# Autodesk Inventor assembly: CN3065 Solar Charger board
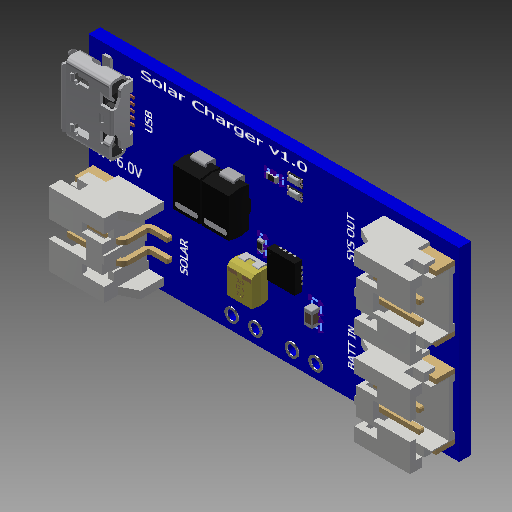
[picture p0: Inventor's stored thumbnail of the model, 512x512]
Saved by Autodesk Inventor 2018 (Build 220112000, 112)
## iProperties
Created: 2019-03-28
Part Number: CN3065 Solar Charger board
Document SubType Name: Assembly
Designer: ZEUSLAP
Author: ZEUSLAP
## Documents named in this file (11)
- C:\Users\ZEUSLAP\YandexDisk\Inventor\solar_harvester_145x145\parts\CN3065 Solar Charger board\CN3065 Solar Charger board.iam
- C:\Users\ZEUSLAP\YandexDisk\Inventor\solar_harvester_145x145\parts\CN3065 Solar Charger board\parts\board.ipt
- C:\Users\ZEUSLAP\YandexDisk\Inventor\solar_harvester_145x145\parts\CN3065 Solar Charger board\parts\micro USB.ipt
- C:\Users\ZEUSLAP\YandexDisk\Inventor\solar_harvester_145x145\parts\CN3065 Solar Charger board\parts\S2B-PH-SM4-TB.ipt
- C:\Users\ZEUSLAP\YandexDisk\Inventor\solar_harvester_145x145\parts\CN3065 Solar Charger board\parts\Diode SMA.ipt
- C:\Users\ZEUSLAP\YandexDisk\Inventor\solar_harvester_145x145\parts\CN3065 Solar Charger board\parts\Tant Cap SMD size B _ 3528-21.ipt
- C:\Users\ZEUSLAP\YandexDisk\Inventor\solar_harvester_145x145\parts\CN3065 Solar Charger board\parts\QFN-16 (3x3).ipt
- C:\Users\ZEUSLAP\YandexDisk\Inventor\solar_harvester_145x145\parts\CN3065 Solar Charger board\parts\CAPC-0603-T0.9-BN.ipt
- C:\Users\ZEUSLAP\YandexDisk\Inventor\solar_harvester_145x145\parts\CN3065 Solar Charger board\parts\RESC-0402.ipt
- C:\Users\ZEUSLAP\YandexDisk\Inventor\solar_harvester_145x145\parts\CN3065 Solar Charger board\parts\0603 LED v7.ipt
- C:\Users\ZEUSLAP\YandexDisk\Inventor\solar_harvester_145x145\parts\CN3065 Solar Charger board\parts\hole_plating.ipt
## Components (22 placed, 10 different names)
1. board:1 — Mate:4, Angle:1, Mate:7, Mate:8, Mate:9, Mate:10, Mate:11, Angle:2, Angle:3, Angle:4, Flush:1, Flush:2, Flush:3, Flush:4, Flush:5, Flush:6, Mate:12, Mate:13, Angle:5, Angle:6, Mate:14, Mate:15, Flush:7, Mate:17, Angle:7, Mate:18, Mate:19, Mate:20, Angle:8, Flush:8, Mate:22, Angle:9, Mate:25, Angle:10, Flush:9, Mate:27, Angle:11, Mate:30, Mate:31, Angle:12, Flush:11, Mate:34, Mate:35, Mate:36, Mate:37, Mate:38, Mate:39, Mate:40, Mate:41, Mate:42, Mate:44, Mate:45, Mate:46, Mate:47, Mate:48, Mate:49, Mate:50
2. micro USB:1 — Mate:4, Angle:1, Mate:7, Mate:8
3. S2B-PH-SM4-TB:1 — Mate:9, Angle:2, Flush:1, Flush:3
4. S2B-PH-SM4-TB:2 — Mate:10, Angle:4, Flush:5, Flush:6
5. S2B-PH-SM4-TB:3 — Mate:11, Angle:3, Flush:2, Flush:4
6. Diode SMA:1 — Mate:13, Angle:6, Mate:15, Mate:16, Mate:26, Mate:28
7. Diode SMA:2 — Mate:12, Angle:5, Mate:14, Flush:7, Mate:16
8. Tant Cap SMD size B _ 3528-21:1 — Mate:17, Angle:7, Mate:18, Mate:19, Mate:21, Mate:29
9. QFN-16 (3x3):1 — Mate:20, Angle:8, Mate:21, Flush:8, Mate:23, Mate:24
10. CAPC-0603-T0.9-BN:1 — Mate:22, Angle:9, Mate:23, Mate:24
11. RESC-0402:1 — Mate:25, Angle:10, Flush:9, Mate:26, Mate:33
12. RESC-0402:2 — Mate:27, Angle:11, Mate:28, Mate:29
13. 0603 LED v7:1 — Mate:31, Mate:32, Flush:10
14. 0603 LED v7:2 — Mate:30, Mate:32, Flush:10, Angle:12, Flush:11, Mate:33
15. hole_plating:1 — Mate:36, Mate:41
16. hole_plating:2 — Mate:37, Mate:40
17. hole_plating:3 — Mate:35, Mate:38
18. hole_plating:4 — Mate:34, Mate:39
19. hole_plating:5 — Mate:42, Mate:47
20. hole_plating:6 — Mate:46, Mate:49
21. hole_plating:7 — Mate:44, Mate:50
22. hole_plating:8 — Mate:45, Mate:48
## Relationships (67: Mate 44, Angle 12, Flush 11)
- Mate:4: board:1 ↔ micro USB:1
- Angle:1 (180 deg): board:1 ↔ micro USB:1
- Mate:7 (1 mm): board:1 ↔ micro USB:1
- Mate:8: board:1 ↔ micro USB:1
- Mate:9: board:1 ↔ S2B-PH-SM4-TB:1
- Mate:10: board:1 ↔ S2B-PH-SM4-TB:2
- Mate:11: board:1 ↔ S2B-PH-SM4-TB:3
- Angle:2 (0 deg): board:1 ↔ S2B-PH-SM4-TB:1
- Angle:3 (180 deg): board:1 ↔ S2B-PH-SM4-TB:3
- Angle:4 (180 deg): board:1 ↔ S2B-PH-SM4-TB:2
- Flush:1 (0.5 mm): board:1 ↔ S2B-PH-SM4-TB:1
- Flush:2 (0.5 mm): board:1 ↔ S2B-PH-SM4-TB:3
- Flush:3 (1 mm): board:1 ↔ S2B-PH-SM4-TB:1
- Flush:4 (1 mm): board:1 ↔ S2B-PH-SM4-TB:3
- Flush:5 (0.5 mm): board:1 ↔ S2B-PH-SM4-TB:2
- Flush:6 (0.5 mm): board:1 ↔ S2B-PH-SM4-TB:2
- Mate:12: board:1 ↔ Diode SMA:2
- Mate:13: board:1 ↔ Diode SMA:1
- Angle:5 (0 deg): board:1 ↔ Diode SMA:2
- Angle:6 (0 deg): board:1 ↔ Diode SMA:1
- Mate:14 (-5 mm): board:1 ↔ Diode SMA:2
- Mate:15 (-5 mm): board:1 ↔ Diode SMA:1
- Flush:7 (-11.5 mm): board:1 ↔ Diode SMA:2
- Mate:16 (0.2 mm): Diode SMA:1 ↔ Diode SMA:2
- Mate:17: board:1 ↔ Tant Cap SMD size B _ 3528-21:1
- Angle:7 (0 deg): board:1 ↔ Tant Cap SMD size B _ 3528-21:1
- Mate:18 (17 mm): board:1 ↔ Tant Cap SMD size B _ 3528-21:1
- Mate:19 (-5 mm): board:1 ↔ Tant Cap SMD size B _ 3528-21:1
- Mate:20: board:1 ↔ QFN-16 (3x3):1
- Angle:8 (180 deg): board:1 ↔ QFN-16 (3x3):1
- Mate:21 (0.5 mm): Tant Cap SMD size B _ 3528-21:1 ↔ QFN-16 (3x3):1
- Flush:8 (7.5 mm): board:1 ↔ QFN-16 (3x3):1
- Mate:22: board:1 ↔ CAPC-0603-T0.9-BN:1
- Angle:9 (90 deg): board:1 ↔ CAPC-0603-T0.9-BN:1
- Mate:23 (1 mm): QFN-16 (3x3):1 ↔ CAPC-0603-T0.9-BN:1
- Mate:24 (0.5 mm): QFN-16 (3x3):1 ↔ CAPC-0603-T0.9-BN:1
- Mate:25: board:1 ↔ RESC-0402:1
- Angle:10 (270 deg): board:1 ↔ RESC-0402:1
- Flush:9 (3 mm): board:1 ↔ RESC-0402:1
- Mate:26 (2 mm): Diode SMA:1 ↔ RESC-0402:1
- Mate:27: board:1 ↔ RESC-0402:2
- Angle:11 (90 deg): board:1 ↔ RESC-0402:2
- Mate:28 (1 mm): Diode SMA:1 ↔ RESC-0402:2
- Mate:29 (1 mm): Tant Cap SMD size B _ 3528-21:1 ↔ RESC-0402:2
- Mate:30: board:1 ↔ 0603 LED v7:2
- Mate:31: board:1 ↔ 0603 LED v7:1
- Mate:32 (0.5 mm): 0603 LED v7:1 ↔ 0603 LED v7:2
- Flush:10: 0603 LED v7:1 ↔ 0603 LED v7:2
- Angle:12 (180 deg): board:1 ↔ 0603 LED v7:2
- Flush:11 (-2 mm): board:1 ↔ 0603 LED v7:2
- Mate:33 (1 mm): RESC-0402:1 ↔ 0603 LED v7:2
- Mate:34: board:1 ↔ hole_plating:4
- Mate:35: board:1 ↔ hole_plating:3
- Mate:36: board:1 ↔ hole_plating:1
- Mate:37: board:1 ↔ hole_plating:2
- Mate:38: board:1 ↔ hole_plating:3
- Mate:39: board:1 ↔ hole_plating:4
- Mate:40: board:1 ↔ hole_plating:2
- Mate:41: board:1 ↔ hole_plating:1
- Mate:42: board:1 ↔ hole_plating:5
- Mate:44: board:1 ↔ hole_plating:7
- Mate:45: board:1 ↔ hole_plating:8
- Mate:46: board:1 ↔ hole_plating:6
- Mate:47: board:1 ↔ hole_plating:5
- Mate:48: board:1 ↔ hole_plating:8
- Mate:49: board:1 ↔ hole_plating:6
- Mate:50: board:1 ↔ hole_plating:7
